# Autodesk Inventor assembly: Engine Assembly
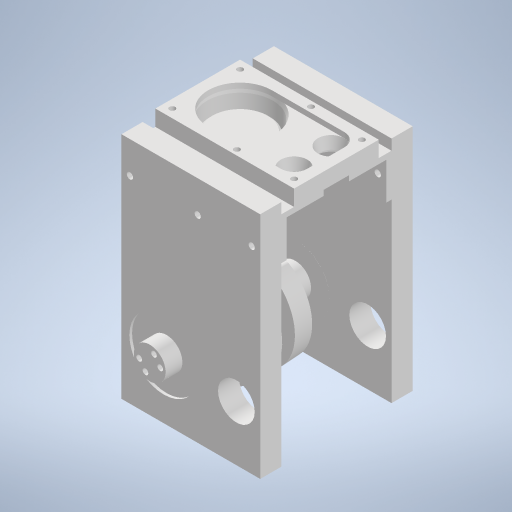
[picture p0: Inventor's stored thumbnail of the model, 512x512]
Saved by Autodesk Inventor 2023 (Build 270158000, 158)
## iProperties
Created: 2022-12-22
Part Number: Engine Assembly
Document SubType Name: Assembly
Designer: tgr41
Author: tgr41
## Documents named in this file (6)
- C:\Users\tgr41\OneDrive\Documents\Repositories\Steam-Engine\2 Inch V3\Engine Assembly.iam
- C:\Users\tgr41\OneDrive\Documents\Repositories\Steam-Engine\2 Inch V3\Piston Subassembly.iam
- C:\Users\tgr41\OneDrive\Documents\Repositories\Steam-Engine\2 Inch V3\Connecting Rod.iam
- C:\Users\tgr41\OneDrive\Documents\Repositories\Steam-Engine\2 Inch V3\CrankShaft Main Bearing.ipt
- C:\Users\tgr41\OneDrive\Documents\Repositories\Steam-Engine\2 Inch V3\Head Cylinder and Frame Subassembly.iam
- C:\Users\tgr41\OneDrive\Documents\Repositories\Steam-Engine\2 Inch V3\Crankshaft Subassembly.iam
## Components (7 placed, 5 different names)
1. Piston Subassembly:1 [sub-assembly] — Mate:1, Mate:2, Mate:3, Flush:1
2. Connecting Rod:1 [sub-assembly] — Mate:1, Mate:2, Mate:4, Mate:5, Mate:6, Mate:7
3. Head Cylinder and Frame Subassembly:1 [sub-assembly] — Mate:3, Angle:1, Flush:1, Mate:11, Mate:12, Mate:13
4. Crankshaft Subassembly:1 [sub-assembly] — Mate:6, Mate:7, Angle:1, Mate:8, Mate:9
5. Crankshaft Subassembly:2 [sub-assembly] — Mate:4, Mate:5, Mate:8, Mate:10
6. CrankShaft Main Bearing:1 — Mate:9, Mate:11, Mate:13
7. CrankShaft Main Bearing:2 — Mate:10, Mate:12
## Relationships (15: Mate 13, Angle 1, Flush 1)
- Mate:1: Piston Subassembly:1 ↔ Connecting Rod:1
- Mate:2: Piston Subassembly:1 ↔ Connecting Rod:1
- Mate:3: Piston Subassembly:1 ↔ Head Cylinder and Frame Subassembly:1
- Mate:4: Connecting Rod:1 ↔ Crankshaft Subassembly:2
- Mate:5: Connecting Rod:1 ↔ Crankshaft Subassembly:2
- Mate:6: Connecting Rod:1 ↔ Crankshaft Subassembly:1
- Mate:7: Connecting Rod:1 ↔ Crankshaft Subassembly:1
- Angle:1 (0 deg): Head Cylinder and Frame Subassembly:1 ↔ Crankshaft Subassembly:1
- Mate:8: Crankshaft Subassembly:1 ↔ Crankshaft Subassembly:2
- Flush:1: Piston Subassembly:1 ↔ Head Cylinder and Frame Subassembly:1
- Mate:9: Crankshaft Subassembly:1 ↔ CrankShaft Main Bearing:1
- Mate:10: Crankshaft Subassembly:2 ↔ CrankShaft Main Bearing:2
- Mate:11: Head Cylinder and Frame Subassembly:1 ↔ CrankShaft Main Bearing:1
- Mate:12: Head Cylinder and Frame Subassembly:1 ↔ CrankShaft Main Bearing:2
- Mate:13: Head Cylinder and Frame Subassembly:1 ↔ CrankShaft Main Bearing:1
